# Autodesk Inventor assembly: steering assembly v1
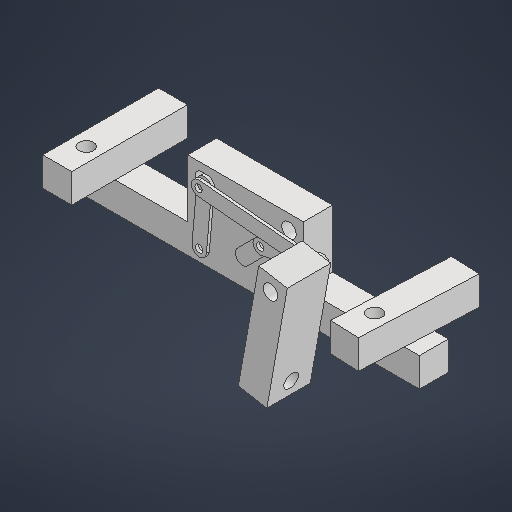
[picture p0: Inventor's stored thumbnail of the model, 512x512]
Saved by Autodesk Inventor 2026.1 (Build 301233000, 233)
## iProperties
Created: 2026-06-10
Part Number: steering assembly v1
Document SubType Name: Assembly
Designer: share
Author: share
## Documents named in this file (8)
- C:\Users\share\OneDrive\Documents\Personal Projects\GOGO Kart\CAD\GOGO_KART_FSAE\Shareef\Suspension Parts\Steering\steering assembly v1.iam
- C:\Users\share\OneDrive\Documents\Personal Projects\GOGO Kart\CAD\GOGO_KART_FSAE\Shareef\Suspension Parts\Steering\center block.ipt
- C:\Users\share\OneDrive\Documents\Personal Projects\GOGO Kart\CAD\GOGO_KART_FSAE\Shareef\Suspension Parts\Steering\main rack connection.ipt
- C:\Users\share\OneDrive\Documents\Personal Projects\GOGO Kart\CAD\GOGO_KART_FSAE\Shareef\Suspension Parts\Steering\arm.ipt
- C:\Users\share\OneDrive\Documents\Personal Projects\GOGO Kart\CAD\GOGO_KART_FSAE\Shareef\Suspension Parts\Steering\arm 1.ipt
- C:\Users\share\OneDrive\Documents\Personal Projects\GOGO Kart\CAD\GOGO_KART_FSAE\Shareef\Suspension Parts\Steering\arm 2.ipt
- C:\Users\share\OneDrive\Documents\Personal Projects\GOGO Kart\CAD\GOGO_KART_FSAE\Shareef\Suspension Parts\Steering\knuckle.ipt
- C:\Users\share\OneDrive\Documents\Personal Projects\GOGO Kart\CAD\GOGO_KART_FSAE\Shareef\Suspension Parts\Steering\tie rod.ipt
## Components (9 placed, 7 different names)
1. center block:1 — Insert:7, Insert:8, Insert:9, Flush:1, Flush:2, Flush:3, Insert:10, Insert:11
2. main rack connection:1 — Insert:3, Insert:7
3. arm:1 — Insert:4, Insert:8
4. arm 1:1 — Insert:3, Insert:4, Insert:6
5. arm 2:1 — Insert:6, Mate:1, Insert:12
6. arm:2 — Mate:1, Insert:9
7. knuckle:1 — Insert:11
8. knuckle:2 — Insert:10
9. tie rod:1 — Insert:12
## Relationships (13: Insert 9, Flush 3, Mate 1)
- Insert:3: main rack connection:1 ↔ arm 1:1
- Insert:4: arm:1 ↔ arm 1:1
- Insert:6: arm 1:1 ↔ arm 2:1
- Mate:1: arm 2:1 ↔ arm:2
- Insert:7: center block:1 ↔ main rack connection:1
- Insert:8: center block:1 ↔ arm:1
- Insert:9: center block:1 ↔ arm:2
- Flush:1: center block:1
- Flush:2: center block:1
- Flush:3: center block:1
- Insert:10: center block:1 ↔ knuckle:2
- Insert:11: center block:1 ↔ knuckle:1
- Insert:12: arm 2:1 ↔ tie rod:1
